# Autodesk Inventor assembly: 000.005 - Блок АКБ
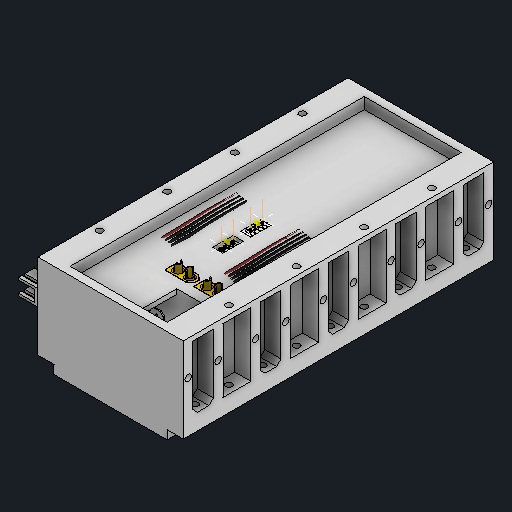
[picture p0: Inventor's stored thumbnail of the model, 512x512]
Saved by Autodesk Inventor 2025 (Build 290162000, 162)
## iProperties
Created: 2024-08-02
Part Number: 000.005 - Блок АКБ
Document SubType Name: Assembly
Designer: IvanPetrov
Author: IvanPetrov
## Documents named in this file (7)
- D:\Projects\OmniBot\design\000.005 - Блок АКБ.iam
- D:\Projects\OmniBot\design\000.005.001 - Корпус.ipt
- D:\Projects\OmniBot\design\standart_components\NUCLEO.ipt
- D:\Projects\OmniBot\design\standart_components\Bosch Relay 12Vdc - 30A SPST.ipt
- D:\Projects\OmniBot\design\standart_components\XT60FemaleConnector.ipt
- D:\Projects\OmniBot\design\standart_components\connectrs\JST - XH - Thru (V) - 4Pin - 2.54mm.ipt
- D:\Projects\OmniBot\design\standart_components\OrangePi 5 Plus LTS\000.005.002 - Кабель канал.ipt
## Components (9 placed, 6 different names)
1. 000.005.001 - Корпус:1 — Касательность:2, Угол:2, Совмещение:3, Совмещение:4, Совмещение:5, Совмещение:6, Совмещение:7, Совмещение:8, Заподлицо:4, Совмещение:10, Угол:3, Совмещение:12, Заподлицо:6
2. NUCLEO:1 — Касательность:2, Угол:2, Заподлицо:1, Совмещение:1, Совмещение:2, Совмещение:3, Совмещение:10
3. NUCLEO:2 — Заподлицо:1, Совмещение:1, Совмещение:2
4. Bosch Relay 12Vdc - 30A SPST:1 — Совмещение:4, Совмещение:5, Совмещение:6
5. XT60FemaleConnector:1 — Совмещение:7, Совмещение:8, Совмещение:9, Заподлицо:2, Заподлицо:3
6. XT60FemaleConnector:2 — Совмещение:9, Заподлицо:2, Заподлицо:3, Заподлицо:4
7. JST - XH - Thru (V) - 4Pin - 2.54mm:1 — Заподлицо:5, Совмещение:11
8. JST - XH - Thru (V) - 4Pin - 2.54mm:2 — Угол:3, Заподлицо:5, Совмещение:11
9. 000.005.002 - Кабель канал:1 — Совмещение:12, Заподлицо:6
## Relationships (21: Mate 12, Flush 6, Angle 2, Tangent 1)
- Касательность:2 [Tangent]: 000.005.001 - Корпус:1 ↔ NUCLEO:1
- Угол:2 [Angle] (0 deg): 000.005.001 - Корпус:1 ↔ NUCLEO:1
- Заподлицо:1 [Flush]: NUCLEO:1 ↔ NUCLEO:2
- Совмещение:1 [Mate] (20 mm): NUCLEO:1 ↔ NUCLEO:2
- Совмещение:2 [Mate]: NUCLEO:1 ↔ NUCLEO:2
- Совмещение:3 [Mate]: 000.005.001 - Корпус:1 ↔ NUCLEO:1
- Совмещение:4 [Mate]: 000.005.001 - Корпус:1 ↔ Bosch Relay 12Vdc - 30A SPST:1
- Совмещение:5 [Mate]: 000.005.001 - Корпус:1 ↔ Bosch Relay 12Vdc - 30A SPST:1
- Совмещение:6 [Mate]: 000.005.001 - Корпус:1 ↔ Bosch Relay 12Vdc - 30A SPST:1
- Совмещение:7 [Mate] (2 mm): 000.005.001 - Корпус:1 ↔ XT60FemaleConnector:1
- Совмещение:8 [Mate] (1.5 mm): 000.005.001 - Корпус:1 ↔ XT60FemaleConnector:1
- Совмещение:9 [Mate] (2 mm): XT60FemaleConnector:1 ↔ XT60FemaleConnector:2
- Заподлицо:2 [Flush]: XT60FemaleConnector:1 ↔ XT60FemaleConnector:2
- Заподлицо:3 [Flush]: XT60FemaleConnector:1 ↔ XT60FemaleConnector:2
- Заподлицо:4 [Flush]: 000.005.001 - Корпус:1 ↔ XT60FemaleConnector:2
- Совмещение:10 [Mate] (1 mm): 000.005.001 - Корпус:1 ↔ NUCLEO:1
- Угол:3 [Angle] (0 deg): 000.005.001 - Корпус:1 ↔ JST - XH - Thru (V) - 4Pin - 2.54mm:2
- Заподлицо:5 [Flush]: JST - XH - Thru (V) - 4Pin - 2.54mm:1 ↔ JST - XH - Thru (V) - 4Pin - 2.54mm:2
- Совмещение:11 [Mate] (5 mm): JST - XH - Thru (V) - 4Pin - 2.54mm:1 ↔ JST - XH - Thru (V) - 4Pin - 2.54mm:2
- Совмещение:12 [Mate]: 000.005.001 - Корпус:1 ↔ 000.005.002 - Кабель канал:1
- Заподлицо:6 [Flush]: 000.005.001 - Корпус:1 ↔ 000.005.002 - Кабель канал:1
